# Autodesk Inventor assembly: richHolderSuppourt
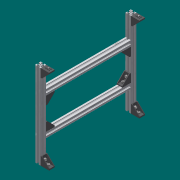
[picture p0: Inventor's stored thumbnail of the model, 180x180]
Saved by Autodesk Inventor 2016 SP1 (Build 200210100, 210)
## iProperties
Created: 2016-02-08
Part Number: richHolderSuppourt
Document SubType Name: Assembly
Designer: Sawaiz
Author: Sawaiz
## Documents named in this file (5)
- C:\Users\sawai\OneDrive\projects\modularRICHFrame\frame\richHolderSuppourt.iam
- C:\Users\sawai\OneDrive\projects\modularRICHFrame\hardware\angleBracket.iam
- C:\Users\sawai\OneDrive\projects\modularRICHFrame\frame\hfs5-2020Height.ipt
- C:\Users\sawai\OneDrive\projects\modularRICHFrame\frame\hfs5-2020Width.ipt
- C:\Users\sawai\OneDrive\projects\modularRICHFrame\modularRICHFrame.xlsx
## Components (12 placed, 3 different names)
1. angleBracket:1 [sub-assembly] — Flush:26, Flush:27, Mate:13, Flush:47
2. angleBracket:2 [sub-assembly] — Flush:28, Flush:29, Mate:14
3. angleBracket:3 [sub-assembly] — Symmetry:3, Flush:24, Flush:25, Mate:15, Flush:47
4. angleBracket:4 [sub-assembly] — Symmetry:3, Mate:12, Flush:22, Flush:23
5. angleBracket:5 [sub-assembly] — Flush:6, Flush:7, Flush:10, Flush:12, Flush:32, Flush:37, Flush:38, Flush:39, Flush:41, Mate:17, Flush:45, Flush:46
6. angleBracket:6 [sub-assembly] — Flush:6, Flush:10, Flush:13, Flush:33, Flush:36, Flush:37, Flush:40, Flush:44, Mate:19
7. angleBracket:7 [sub-assembly] — Flush:5, Flush:7, Flush:9, Flush:12, Flush:31, Flush:35, Flush:41, Flush:43, Mate:18
8. angleBracket:8 [sub-assembly] — Flush:5, Flush:9, Flush:13, Flush:30, Flush:35, Flush:36, Flush:40, Mate:16, Flush:42
9. hfs5-2020Height:1 — Flush:26, Flush:27, Flush:28, Flush:29, Mate:13, Mate:14, Symmetry:4, Flush:34, Symmetry:5, Mate:18
10. hfs5-2020Height:2 — Mate:12, Flush:22, Flush:23, Flush:24, Flush:25, Symmetry:4, Flush:34, Mate:15, Symmetry:5, Flush:46, Mate:19
11. hfs5-2020Width:1 — Flush:30, Flush:33, Flush:38, Mate:16, Flush:42, Flush:44, Symmetry:6, Mate:20
12. hfs5-2020Width:2 — Flush:31, Flush:32, Flush:39, Mate:17, Flush:43, Flush:45, Symmetry:6, Mate:20
## Relationships (46: Flush 33, Mate 9, Symmetry 4)
- Flush:5: angleBracket:7 ↔ angleBracket:8
- Flush:6: angleBracket:5 ↔ angleBracket:6
- Flush:7: angleBracket:5 ↔ angleBracket:7
- Flush:9: angleBracket:7 ↔ angleBracket:8
- Flush:10: angleBracket:5 ↔ angleBracket:6
- Flush:12: angleBracket:5 ↔ angleBracket:7
- Flush:13: angleBracket:6 ↔ angleBracket:8
- Symmetry:3: angleBracket:3 ↔ angleBracket:4
- Mate:12: angleBracket:4 ↔ hfs5-2020Height:2
- Flush:22: angleBracket:4 ↔ hfs5-2020Height:2
- Flush:23: angleBracket:4 ↔ hfs5-2020Height:2
- Flush:24: angleBracket:3 ↔ hfs5-2020Height:2
- Flush:25: angleBracket:3 ↔ hfs5-2020Height:2
- Flush:26: angleBracket:1 ↔ hfs5-2020Height:1
- Flush:27: angleBracket:1 ↔ hfs5-2020Height:1
- Flush:28: angleBracket:2 ↔ hfs5-2020Height:1
- Flush:29: angleBracket:2 ↔ hfs5-2020Height:1
- Flush:30: angleBracket:8 ↔ hfs5-2020Width:1
- Flush:31: angleBracket:7 ↔ hfs5-2020Width:2
- Flush:32: angleBracket:5 ↔ hfs5-2020Width:2
- Flush:33: angleBracket:6 ↔ hfs5-2020Width:1
- Mate:13: angleBracket:1 ↔ hfs5-2020Height:1
- Mate:14: angleBracket:2 ↔ hfs5-2020Height:1
- Symmetry:4: hfs5-2020Height:1 ↔ hfs5-2020Height:2
- Flush:34: hfs5-2020Height:1 ↔ hfs5-2020Height:2
- Mate:15: angleBracket:3 ↔ hfs5-2020Height:2
- Symmetry:5: hfs5-2020Height:1 ↔ hfs5-2020Height:2
- Flush:35: angleBracket:7 ↔ angleBracket:8
- Flush:36: angleBracket:6 ↔ angleBracket:8
- Flush:37: angleBracket:5 ↔ angleBracket:6
- Flush:38: angleBracket:5 ↔ hfs5-2020Width:1
- Flush:39: angleBracket:5 ↔ hfs5-2020Width:2
- Flush:40: angleBracket:6 ↔ angleBracket:8
- Mate:16: angleBracket:8 ↔ hfs5-2020Width:1
- Flush:41: angleBracket:5 ↔ angleBracket:7
- Mate:17: angleBracket:5 ↔ hfs5-2020Width:2
- Flush:42: angleBracket:8 ↔ hfs5-2020Width:1
- Flush:43: angleBracket:7 ↔ hfs5-2020Width:2
- Flush:44: angleBracket:6 ↔ hfs5-2020Width:1
- Flush:45: angleBracket:5 ↔ hfs5-2020Width:2
- Flush:46: angleBracket:5 ↔ hfs5-2020Height:2
- Mate:18: angleBracket:7 ↔ hfs5-2020Height:1
- Symmetry:6: hfs5-2020Width:1 ↔ hfs5-2020Width:2
- Mate:19: angleBracket:6 ↔ hfs5-2020Height:2
- Flush:47: angleBracket:1 ↔ angleBracket:3
- Mate:20 (111.2 mm): hfs5-2020Width:1 ↔ hfs5-2020Width:2
## Named parameters: frameAcrylicThickness = 9.525 mm, internalAcrylicThickness = 6.35 mm, aerogelThickness = 30 mm, aerogelWidth = 110 mm, aerogelHeight = 110 mm, height = 300 mm, width = 300 mm, depth = 500 mm, mirrorAngle = 5 deg, detectorWidth = 52 mm, detectorHeight = 52 mm, mirrorThickness = 3.175 mm, fresnelThickness = 0.1 mm, grooveDensity = 100, focalLength = 76.2 mm, ior = 1.49, centerThickness = 1.524 mm, fresnelAngle = 90 deg, fresnelEffectiveDiameter = 152.4 mm, oRingWidth = 1.5875 mm, sensorHolderDepth = 19.05 mm, aerogelClearence = 3.175 mm, backplanePCBWidth = 76.2 mm, backplanePCBHeight = 76.2 mm, backplaneHoleOffsett = 6.35 mm, backplanePostionOffsett = 12.7 mm, moduleSlotClearence = 0.79375 mm, testMountLength = 500 mm, testMountWidth = 300 mm, testMountHeight = 300 mm, facingGasketThickness = 1.5875 mm, facingThickness = 12.7 mm
